# Autodesk Inventor assembly: montagem-arcade2
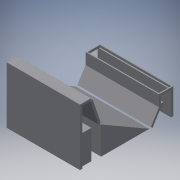
[picture p0: Inventor's stored thumbnail of the model, 180x180]
Saved by Autodesk Inventor 2016 (Build 200138000, 138)
## iProperties
Created: 2017-06-05
Part Number: montagem-arcade2
Material: Genérico
Document SubType Name: Assembly
Designer: Fabio
Author: Fabio
## Documents named in this file (16)
- C:\dev\arcade\montagem-arcade2.iam
- C:\dev\arcade\lateral.ipt
- C:\dev\arcade\coneTela.ipt
- C:\dev\arcade\traseira.ipt
- C:\dev\arcade\BASE.ipt
- C:\dev\arcade\frente inferior.ipt
- C:\dev\arcade\controles.ipt
- C:\dev\arcade\junta controler.ipt
- C:\dev\arcade\fechamento superior.ipt
- C:\dev\arcade\letreiro.ipt
- C:\dev\arcade\fechamento inferior.ipt
- C:\dev\arcade\junta auto falante.ipt
- C:\dev\arcade\placa auto falante.ipt
- C:\dev\arcade\speaker.ipt
- C:\dev\arcade\power supply.ipt
- C:\dev\arcade\sound amplifier.ipt
## Components (17 placed, 15 different names)
1. lateral:1 — Coincidência:2, Alinhamento:1, Alinhamento:4, Mate:4, Mate:6
2. lateral:2 — Coincidência:1, Alinhamento:2, Alinhamento:3, Mate:3, Flush:5, Flush:6, Mate:9, Mate:12, Mate:15
3. coneTela:1 — Coincidência:1, Coincidência:2, Alinhamento:1, Alinhamento:2, Alinhamento:3, Alinhamento:4
4. traseira:1 — Mate:3, Flush:5, Flush:6, Mate:4, Mate:5, Flush:7, Mate:7, Mate:14, Flush:10
5. BASE:1 — Mate:5, Flush:7, Mate:6, Mate:7, Mate:8, Flush:8, Alinhamento:21, Coincidência:23, Alinhamento:22, Alinhamento:23, Coincidência:24, Alinhamento:24
6. frente inferior:1 — Mate:8, Flush:8, Mate:9, Mate:10, Mate:11
7. junta controler:1 — Mate:10, Mate:11, Mate:12, Mate:13, Flush:9
8. controles:1 — Mate:13, Flush:9
9. fechamento superior:1 — Mate:14, Flush:10, Mate:15, Flush:11, Flush:12, Mate:16
10. letreiro:1 — Flush:11, Flush:12, Mate:16, Flush:13, Mate:17, Flush:14
11. fechamento inferior:1 — Flush:13, Mate:17, Flush:14, Coincidência:18, Coincidência:19, Alinhamento:15, Alinhamento:16
12. junta auto falante:1 — Coincidência:18, Coincidência:19, Alinhamento:15, Coincidência:20
13. placa auto falante:1 — Coincidência:20, Alinhamento:16, Coincidência:21, Alinhamento:17, Alinhamento:18, Coincidência:22, Alinhamento:19, Alinhamento:20
14. speaker:1 — Coincidência:22, Alinhamento:19, Alinhamento:20
15. speaker:2 — Coincidência:21, Alinhamento:17, Alinhamento:18
16. power supply:1 — Alinhamento:21, Coincidência:23, Alinhamento:22
17. sound amplifier:1 — Alinhamento:23, Coincidência:24, Alinhamento:24
## Relationships (48: Mate 24, Flush 24)
- Coincidência:1 [Mate]: lateral:2 ↔ coneTela:1
- Coincidência:2 [Mate]: lateral:1 ↔ coneTela:1
- Alinhamento:1 [Flush] (-110 mm): lateral:1 ↔ coneTela:1
- Alinhamento:2 [Flush] (-105 mm): lateral:2 ↔ coneTela:1
- Alinhamento:3 [Flush] (15 mm): lateral:2 ↔ coneTela:1
- Alinhamento:4 [Flush] (10 mm): lateral:1 ↔ coneTela:1
- Mate:3: lateral:2 ↔ traseira:1
- Flush:5: lateral:2 ↔ traseira:1
- Flush:6 (10 mm): lateral:2 ↔ traseira:1
- Mate:4: lateral:1 ↔ traseira:1
- Mate:5: traseira:1 ↔ BASE:1
- Flush:7: traseira:1 ↔ BASE:1
- Mate:6: lateral:1 ↔ BASE:1
- Mate:7: traseira:1 ↔ BASE:1
- Mate:8: BASE:1 ↔ frente inferior:1
- Flush:8: BASE:1 ↔ frente inferior:1
- Mate:9: lateral:2 ↔ frente inferior:1
- Mate:10: frente inferior:1 ↔ junta controler:1
- Mate:11: frente inferior:1 ↔ junta controler:1
- Mate:12: lateral:2 ↔ junta controler:1
- Mate:13: junta controler:1 ↔ controles:1
- Flush:9: junta controler:1 ↔ controles:1
- Mate:14: traseira:1 ↔ fechamento superior:1
- Flush:10: traseira:1 ↔ fechamento superior:1
- Mate:15: lateral:2 ↔ fechamento superior:1
- Flush:11: fechamento superior:1 ↔ letreiro:1
- Flush:12: fechamento superior:1 ↔ letreiro:1
- Mate:16: fechamento superior:1 ↔ letreiro:1
- Flush:13: letreiro:1 ↔ fechamento inferior:1
- Mate:17: letreiro:1 ↔ fechamento inferior:1
- Flush:14: letreiro:1 ↔ fechamento inferior:1
- Coincidência:18 [Mate]: fechamento inferior:1 ↔ junta auto falante:1
- Coincidência:19 [Mate]: fechamento inferior:1 ↔ junta auto falante:1
- Alinhamento:15 [Flush]: fechamento inferior:1 ↔ junta auto falante:1
- Coincidência:20 [Mate]: junta auto falante:1 ↔ placa auto falante:1
- Alinhamento:16 [Flush]: fechamento inferior:1 ↔ placa auto falante:1
- Coincidência:21 [Mate]: placa auto falante:1 ↔ speaker:2
- Alinhamento:17 [Flush] (20 mm): placa auto falante:1 ↔ speaker:2
- Alinhamento:18 [Flush] (15 mm): placa auto falante:1 ↔ speaker:2
- Coincidência:22 [Mate]: placa auto falante:1 ↔ speaker:1
- Alinhamento:19 [Flush] (15 mm): placa auto falante:1 ↔ speaker:1
- Alinhamento:20 [Flush] (20 mm): placa auto falante:1 ↔ speaker:1
- Alinhamento:21 [Flush]: BASE:1 ↔ power supply:1
- Coincidência:23 [Mate]: BASE:1 ↔ power supply:1
- Alinhamento:22 [Flush]: BASE:1 ↔ power supply:1
- Alinhamento:23 [Flush]: BASE:1 ↔ sound amplifier:1
- Coincidência:24 [Mate]: BASE:1 ↔ sound amplifier:1
- Alinhamento:24 [Flush]: BASE:1 ↔ sound amplifier:1
